# Autodesk Inventor assembly: Forearm2
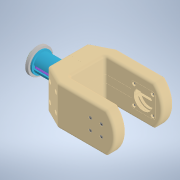
[picture p0: Inventor's stored thumbnail of the model, 180x180]
Saved by Autodesk Inventor 2021 (Build 250183000, 183)
## iProperties
Created: 2020-03-07
Part Number: Forearm2
Document SubType Name: Assembly
Designer: JochenAlt
Author: JochenAlt
## Documents named in this file (7)
- C:\Users\Jochen Alt\Documents\Daten\Projects\MiniBot\CAD\Forearm.iam
- C:\Users\Jochen Alt\Documents\Daten\Projects\MiniBot\CAD\Forearm.ipt
- C:\Users\Jochen Alt\Documents\Daten\Projects\MiniBot\CAD\ForearmShaft.ipt
- C:\Users\Jochen Alt\Documents\Daten\Projects\MiniBot\CAD\extern\bearings\25x32x4\W 61705-2RS1.iam
- C:\Users\Jochen Alt\Documents\Inventor\Content Center Files\R2021\en-US\DIN 912\DIN 912 - M2 x 0.4 x 12 x 11.ipt
- C:\Users\Jochen Alt\Documents\Inventor\Content Center Files\R2021\en-US\DIN 912\DIN 912 - M2 x 0.4 x 20 x 19.ipt
- C:\Users\Jochen Alt\Documents\Inventor\Content Center Files\R2021\en-US\DIN 912\DIN 912 - M2 x 0.4 x 16 x 15.ipt
## Components (22 placed, 6 different names)
1. Forearm:1 — Passend:2, Passend:7, Insert:1, Insert:2, Insert:3, Insert:4, Insert:5, Insert:6, Insert:7, Insert:8, Insert:9, Insert:10, Insert:11, Insert:12, Insert:13, Insert:14, Insert:15, Insert:16
2. ForearmShaft:1 — Passend:2, Passend:3, Passend:4, Passend:5, Passend:6, Passend:7, Mate:8, Mate:9, Mate:10, Mate:11
3. W 61705-2RS1:1 [sub-assembly] — Passend:3, Passend:5
4. W 61705-2RS1:2 [sub-assembly] — Passend:4, Passend:6
5. DIN 912 - replaced by DIN EN ISO 4762 M2 x 12:1 — Insert:1
6. DIN 912 - replaced by DIN EN ISO 4762 M2 x 12:2 — Insert:2
7. DIN 912 - replaced by DIN EN ISO 4762 M2 x 12:3 — Insert:3
8. DIN 912 - replaced by DIN EN ISO 4762 M2 x 12:4 — Insert:4
9. DIN 912 - replaced by DIN EN ISO 4762 M2 x 20:1 — Insert:5
10. DIN 912 - replaced by DIN EN ISO 4762 M2 x 20:2 — Insert:6
11. DIN 912 - replaced by DIN EN ISO 4762 M2 x 20:3 — Insert:7
12. DIN 912 - replaced by DIN EN ISO 4762 M2 x 20:4 — Insert:8
13. DIN 912 - replaced by DIN EN ISO 4762 M2 x 16:1 — Insert:9
14. DIN 912 - replaced by DIN EN ISO 4762 M2 x 16:2 — Insert:10
15. DIN 912 - replaced by DIN EN ISO 4762 M2 x 20:5 — Insert:11
16. DIN 912 - replaced by DIN EN ISO 4762 M2 x 20:6 — Insert:12
17. DIN 912 - replaced by DIN EN ISO 4762 M2 x 20:7 — Insert:13
18. DIN 912 - replaced by DIN EN ISO 4762 M2 x 20:8 — Insert:14
19. DIN 912 - replaced by DIN EN ISO 4762 M2 x 16:3 — Insert:15
20. DIN 912 - replaced by DIN EN ISO 4762 M2 x 16:4 — Insert:16
21. W 61705-2RS1:3 [sub-assembly] — Mate:8, Mate:11
22. W 61705-2RS1:4 [sub-assembly] — Mate:9, Mate:10
## Relationships (26: Insert 16, Mate 10)
- Passend:2 [Mate]: Forearm:1 ↔ ForearmShaft:1
- Passend:3 [Mate]: ForearmShaft:1 ↔ W 61705-2RS1:1
- Passend:4 [Mate]: ForearmShaft:1 ↔ W 61705-2RS1:2
- Passend:5 [Mate]: ForearmShaft:1 ↔ W 61705-2RS1:1
- Passend:6 [Mate]: ForearmShaft:1 ↔ W 61705-2RS1:2
- Passend:7 [Mate]: Forearm:1 ↔ ForearmShaft:1
- Insert:1: Forearm:1 ↔ DIN 912 - replaced by DIN EN ISO 4762 M2 x 12:1
- Insert:2: Forearm:1 ↔ DIN 912 - replaced by DIN EN ISO 4762 M2 x 12:2
- Insert:3: Forearm:1 ↔ DIN 912 - replaced by DIN EN ISO 4762 M2 x 12:3
- Insert:4: Forearm:1 ↔ DIN 912 - replaced by DIN EN ISO 4762 M2 x 12:4
- Insert:5: Forearm:1 ↔ DIN 912 - replaced by DIN EN ISO 4762 M2 x 20:1
- Insert:6: Forearm:1 ↔ DIN 912 - replaced by DIN EN ISO 4762 M2 x 20:2
- Insert:7: Forearm:1 ↔ DIN 912 - replaced by DIN EN ISO 4762 M2 x 20:3
- Insert:8: Forearm:1 ↔ DIN 912 - replaced by DIN EN ISO 4762 M2 x 20:4
- Insert:9: Forearm:1 ↔ DIN 912 - replaced by DIN EN ISO 4762 M2 x 16:1
- Insert:10: Forearm:1 ↔ DIN 912 - replaced by DIN EN ISO 4762 M2 x 16:2
- Insert:11: Forearm:1 ↔ DIN 912 - replaced by DIN EN ISO 4762 M2 x 20:5
- Insert:12: Forearm:1 ↔ DIN 912 - replaced by DIN EN ISO 4762 M2 x 20:6
- Insert:13: Forearm:1 ↔ DIN 912 - replaced by DIN EN ISO 4762 M2 x 20:7
- Insert:14: Forearm:1 ↔ DIN 912 - replaced by DIN EN ISO 4762 M2 x 20:8
- Insert:15: Forearm:1 ↔ DIN 912 - replaced by DIN EN ISO 4762 M2 x 16:3
- Insert:16: Forearm:1 ↔ DIN 912 - replaced by DIN EN ISO 4762 M2 x 16:4
- Mate:8: ForearmShaft:1 ↔ W 61705-2RS1:3
- Mate:9: ForearmShaft:1 ↔ W 61705-2RS1:4
- Mate:10: ForearmShaft:1 ↔ W 61705-2RS1:4
- Mate:11: ForearmShaft:1 ↔ W 61705-2RS1:3
